# Autodesk Inventor assembly: battery_cover
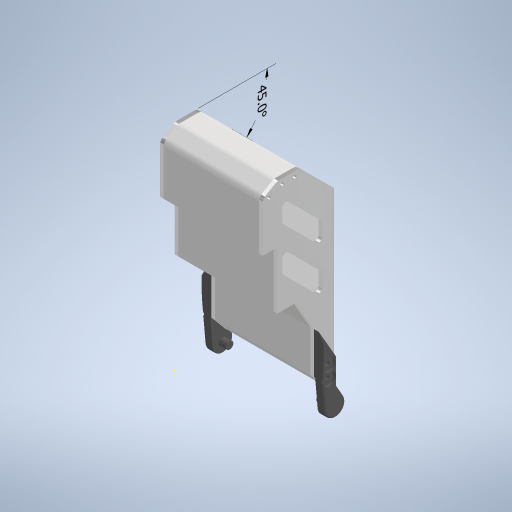
[picture p0: Inventor's stored thumbnail of the model, 512x512]
Saved by Autodesk Inventor 2024.1 (Build 281209000, 209)
## iProperties
Created: 2024-10-11
Part Number: battery_cover
Document SubType Name: Assembly
Designer: hibik
Author: hibik
## Documents named in this file (5)
- C:\Users\hibik\Documents\Robomech\HR\Eglantyne\hard\under_body\battery_cover\battery_cover.iam
- C:\Users\hibik\Documents\Robomech\HR\Eglantyne\hard\under_body\battery_cover\back.ipt
- C:\Users\hibik\Documents\Robomech\HR\Eglantyne\hard\under_body\battery_cover\side_right.ipt
- C:\Users\hibik\Documents\Robomech\HR\Eglantyne\hard\under_body\battery_cover\side_left.ipt
- C:\Users\hibik\Documents\Robomech\HR\Eglantyne\hard\under_body\battery_cover\upper.ipt
## Components (4 placed, 4 different names)
1. side_right:1 — 挿入:1, 挿入:2
2. side_left:1 — 挿入:3, 挿入:4
3. back:1 — フラッシュ:1, メイト:1, フラッシュ:2, 挿入:1, 挿入:2, 挿入:3, 挿入:4
4. upper:1 — フラッシュ:1, メイト:1, フラッシュ:2
## Relationships (7: Insert 4, Flush 2, Mate 1)
- フラッシュ:1 [Flush]: back:1 ↔ upper:1
- メイト:1 [Mate]: back:1 ↔ upper:1
- フラッシュ:2 [Flush]: back:1 ↔ upper:1
- 挿入:1 [Insert]: side_right:1 ↔ back:1
- 挿入:2 [Insert]: side_right:1 ↔ back:1
- 挿入:3 [Insert]: side_left:1 ↔ back:1
- 挿入:4 [Insert]: side_left:1 ↔ back:1
